# Autodesk Inventor assembly: Battery Cage Assembly
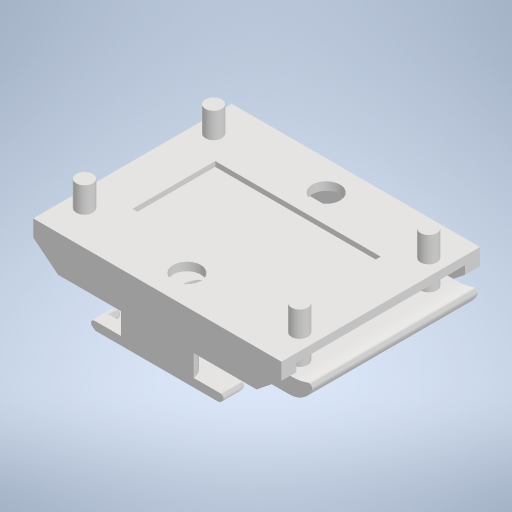
[picture p0: Inventor's stored thumbnail of the model, 512x512]
Saved by Autodesk Inventor 2023 (Build 270158000, 158)
## iProperties
Created: 2022-12-02
Part Number: Battery Cage Assembly
Document SubType Name: Assembly
Designer: cheng
Author: cheng
## Documents named in this file (3)
- C:\Users\cheng\Desktop\4th Year Project\Inventor\Third Assembly\Second Assembly\Battery Cage Assembly.iam
- C:\Users\cheng\Desktop\4th Year Project\Inventor\Third Assembly\Second Assembly\Battery Cage.ipt
- C:\Users\cheng\Desktop\4th Year Project\Inventor\Third Assembly\Second Assembly\Battery Cage Spring Plate.ipt
## Components (2 placed, 2 different names)
1. Battery Cage:1 — Mate:1, Mate:2
2. Battery Cage Spring Plate:1 — Mate:1, Mate:2
## Relationships (2: Mate 2)
- Mate:1: Battery Cage:1 ↔ Battery Cage Spring Plate:1
- Mate:2: Battery Cage:1 ↔ Battery Cage Spring Plate:1
